# Autodesk Inventor assembly: driveAssembly
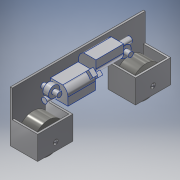
[picture p0: Inventor's stored thumbnail of the model, 180x180]
Saved by Autodesk Inventor 2016 (Build 200138000, 138)
## iProperties
Created: 2015-10-31
Part Number: driveAssembly
Document SubType Name: Assembly
Designer: rossmosier
Author: rossmosier
## Documents named in this file (6)
- C:\Users\rossmosier\Documents\CAD Team\CADTeam\Drive Train\driveAssembly.iam
- C:\Users\rossmosier\Documents\CAD Team\CADTeam\Drive Train\side.ipt
- C:\Users\rossmosier\Documents\CAD Team\CADTeam\Drive Train\driveAssembly\Design Accelerator\Shaft1.iam
- C:\Users\rossmosier\Documents\CAD Team\CADTeam\Parts\bearing.ipt
- C:\Users\rossmosier\Documents\CAD Team\CADTeam\Drive Train\generic wheel.ipt
- C:\Users\rossmosier\Documents\CAD Team\CADTeam\Drive Train\Motor_500RPM.ipt
## Components (9 placed, 5 different names)
1. side:1 — Rigid:1, Rotational:1, Mate:1, Mate:2
2. Shaft:1 [sub-assembly] — Rotational:2, Rotational:4
3. bearing:1 — Rotational:1, Rotational:2
4. bearing:2 — Rigid:1, Rotational:3
5. Shaft:2 [sub-assembly] — Rotational:3
6. generic wheel:1
7. generic wheel:2 — Rotational:4
8. Motor_500RPM:1 — Mate:1
9. Motor_500RPM:2 — Mate:2
## Relationships (7: RevoluteJoint 4, Mate 2, WeldJoint 1)
- Rigid:1 [WeldJoint] (-1.5875 mm): side:1 ↔ bearing:2
- Rotational:1 [RevoluteJoint]: side:1 ↔ bearing:1
- Rotational:2 [RevoluteJoint] (-6.35 mm): Shaft:1 ↔ bearing:1
- Rotational:3 [RevoluteJoint] (-6.35 mm): bearing:2 ↔ Shaft:2
- Rotational:4 [RevoluteJoint] (-25.4 mm): Shaft:1 ↔ generic wheel:2
- Mate:1: side:1 ↔ Motor_500RPM:1
- Mate:2: side:1 ↔ Motor_500RPM:2
